# Autodesk Inventor assembly: hand
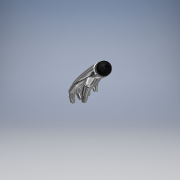
[picture p0: Inventor's stored thumbnail of the model, 180x180]
Saved by Autodesk Inventor 2018 (Build 220112000, 112)
## iProperties
Created: 2020-03-01
Part Number: hand
Document SubType Name: Assembly
Designer: Matt
Author: Matt
## Documents named in this file (2)
- C:\Users\Matt\robot\multibodySim\human\Corpo Humano - ADEBOTT Projetos\hand.iam
- C:\Users\Matt\robot\multibodySim\human\Corpo Humano - ADEBOTT Projetos\01.02.02.03 - Mão direita.ipt
## Components (1 placed, 1 different names)
1. 01.02.02.03 - Mão direita:1 — Tangent:1, Tangent:2, Tangent:3
## Relationships (9: Angle 3, Tangent 3, Flush 2, Mate 1)
- Angle:1 (0 deg)
- Tangent:1: 01.02.02.03 - Mão direita:1
- Angle:2 (0 deg)
- Tangent:2: 01.02.02.03 - Mão direita:1
- Angle:3 (0 deg)
- Tangent:3: 01.02.02.03 - Mão direita:1
- Flush:1 (-22 mm)
- Flush:2 (-22 mm)
- Mate:1 (22 mm)
